# Autodesk Inventor assembly: frame_solid
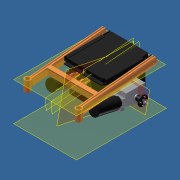
[picture p0: Inventor's stored thumbnail of the model, 180x180]
Saved by Autodesk Inventor 2012 (Build 160160000, 160)
## iProperties
Created: 2012-03-08
Part Number: frame_solid
Document SubType Name: Assembly
Designer: esv
Mass: 83979.9 g
Surface Area: 24308.3 cm^2
Volume: 48170.3 cm^3
Density: 1.7434 g/cm^3
Author: esv
## Documents named in this file (5)
- C:\Users\Edward\Documents\masters\CAD\Invacare\frame_solid.iam
- C:\Users\Edward\Documents\masters\CAD\Invacare\frame assy.iam
- C:\Users\Edward\Documents\masters\CAD\Invacare\motor.ipt
- C:\Users\Edward\Documents\masters\CAD\Invacare\motor_MIR.ipt
- C:\Users\Edward\Documents\masters\CAD\Invacare\lumped batteries.iam
## Components (4 placed, 4 different names)
1. frame assy:1 [sub-assembly] — Flush:1, Angle:1, Flush:6, Mate:10, Mate:11, Mate:12, Mate:13, Mate:14, Mate:15
2. motor:1 — Flush:4, Flush:5, Mate:9
3. motor_MIR:1 — Flush:4, Flush:5, Mate:9, Flush:6, Flush:7, Mate:11
4. lumped batteries:1 [sub-assembly] — Mate:12, Mate:13, Mate:14, Mate:15
## Relationships (13: Mate 7, Flush 5, Angle 1)
- Flush:1: frame assy:1
- Angle:1 (0 deg): frame assy:1
- Flush:4: motor:1 ↔ motor_MIR:1
- Flush:5: motor:1 ↔ motor_MIR:1
- Mate:9 (285.75 mm): motor:1 ↔ motor_MIR:1
- Flush:6 (233.3625 mm): frame assy:1 ↔ motor_MIR:1
- Flush:7 (142.875 mm): motor_MIR:1
- Mate:10: frame assy:1
- Mate:11 (-101.6 mm): frame assy:1 ↔ motor_MIR:1
- Mate:12: frame assy:1 ↔ lumped batteries:1
- Mate:13: frame assy:1 ↔ lumped batteries:1
- Mate:14: frame assy:1 ↔ lumped batteries:1
- Mate:15: frame assy:1 ↔ lumped batteries:1
